# Autodesk Inventor assembly: Assembly_10x_Couplingscanner
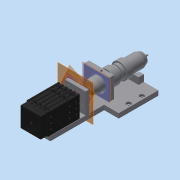
[picture p0: Inventor's stored thumbnail of the model, 180x180]
Saved by Autodesk Inventor 2019.4 (Build 234330000, 330)
## iProperties
Created: 2020-12-14
Part Number: Assembly_10x_Couplingscanner
Document SubType Name: Assembly
Designer: diederichbenedict
Author: diederichbenedict
## Documents named in this file (5)
- C:\Users\diederichbenedict\Dropbox\Dokumente\Promotion\PROJECTS\STORMoChip\GITHUB\CAD\cellSTORM_inverted\Workspace\Assembly_10x_Couplingscanner.iam
- C:\Users\diederichbenedict\Dropbox\Dokumente\Promotion\PROJECTS\STORMoChip\GITHUB\CAD\cellSTORM_inverted\Workspace\00_objectivelens_10x.ipt
- C:\Users\diederichbenedict\Dropbox\Dokumente\Promotion\PROJECTS\STORMoChip\GITHUB\CAD\cellSTORM_inverted\Workspace\00_LASER_640nm.ipt
- C:\Users\diederichbenedict\Dropbox\Dokumente\Promotion\PROJECTS\STORMoChip\GITHUB\CAD\cellSTORM_inverted\Workspace\00_KES400.iam
- C:\Users\diederichbenedict\Dropbox\Dokumente\Promotion\PROJECTS\STORMoChip\GITHUB\CAD\cellSTORM_inverted\Workspace\cellSTORM_inverted_Laser_10x_laserscanner_left.ipt
## Components (5 placed, 4 different names)
1. cellSTORM_inverted_Laser_10x_laserscanner_left:1 — Insert:4, Angle:3, Angle:4, Mate:2, Flush:1, Flush:2
2. 00_objectivelens_10x:1 — Insert:1
3. 00_KES400:1 [sub-assembly] — Insert:2, Insert:4, Angle:2, Mate:1, Angle:3, Flush:1
4. 00_objectivelens_10x:2 — Insert:1, Insert:2
5. 00_LASER_640nm:1 — Mate:1, Angle:4, Mate:2, Flush:2
## Relationships (10: Insert 3, Angle 3, Mate 2, Flush 2)
- Insert:1 (1 mm): 00_objectivelens_10x:1 ↔ 00_objectivelens_10x:2
- Insert:2 (2 mm): 00_KES400:1 ↔ 00_objectivelens_10x:2
- Insert:4: cellSTORM_inverted_Laser_10x_laserscanner_left:1 ↔ 00_KES400:1
- Angle:2 (0 deg): 00_KES400:1
- Mate:1: 00_KES400:1 ↔ 00_LASER_640nm:1
- Angle:3 (180 deg): cellSTORM_inverted_Laser_10x_laserscanner_left:1 ↔ 00_KES400:1
- Angle:4 (0 deg): cellSTORM_inverted_Laser_10x_laserscanner_left:1 ↔ 00_LASER_640nm:1
- Mate:2 (10 mm): cellSTORM_inverted_Laser_10x_laserscanner_left:1 ↔ 00_LASER_640nm:1
- Flush:1: cellSTORM_inverted_Laser_10x_laserscanner_left:1 ↔ 00_KES400:1
- Flush:2 (14 mm): cellSTORM_inverted_Laser_10x_laserscanner_left:1 ↔ 00_LASER_640nm:1
